# Autodesk Inventor assembly: staw
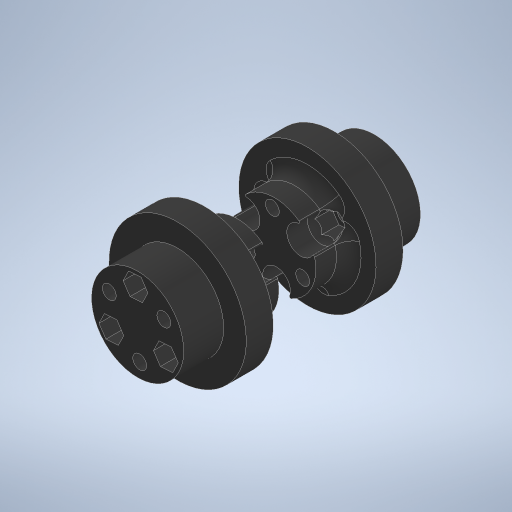
[picture p0: Inventor's stored thumbnail of the model, 512x512]
Saved by Autodesk Inventor 2023 (Build 270158000, 158)
## iProperties
Created: 2023-04-06
Part Number: staw
Document SubType Name: Assembly
Designer: Kamil
Author: Kamil
## Documents named in this file (5)
- C:\Users\Kamil\Desktop\PULPIT\KONARM_2\czlon 3\staw.iam
- C:\Users\Kamil\Desktop\PULPIT\KONARM_2\czlon 3\Os.ipt
- C:\Users\Kamil\Desktop\PULPIT\KONARM_2\czlon 3\Os_lewa.ipt
- C:\Users\Kamil\Desktop\PULPIT\KONARM_2\czlon 3\kółko.ipt
- C:\Users\Kamil\Desktop\PULPIT\KONARM_2\czlon 3\ball bearing(6006).ipt
## Components (6 placed, 4 different names)
1. Os:1 — Zestawiające:1, Zestawiające:2, Zestawiające:3, Zestawiające:12, Zestawiające:13, Zestawiające:15
2. Os_lewa:1 — Zestawiające:1, Zestawiające:2, Zestawiające:3, Zestawiające:10, Zestawiające:11, Zestawiające:16
3. ball bearing(6006):1 — Zestawiające:10, Zestawiające:11, Zestawiające:17
4. ball bearing(6006):2 — Zestawiające:12, Zestawiające:13, Zestawiające:14
5. kółko:2 — Zestawiające:16, Zestawiające:17
6. kółko:3 — Zestawiające:14, Zestawiające:15
## Relationships (11: Mate 11)
- Zestawiające:1 [Mate] (12 mm): Os:1 ↔ Os_lewa:1
- Zestawiające:2 [Mate]: Os:1 ↔ Os_lewa:1
- Zestawiające:3 [Mate]: Os:1 ↔ Os_lewa:1
- Zestawiające:10 [Mate]: Os_lewa:1 ↔ ball bearing(6006):1
- Zestawiające:11 [Mate]: Os_lewa:1 ↔ ball bearing(6006):1
- Zestawiające:12 [Mate]: Os:1 ↔ ball bearing(6006):2
- Zestawiające:13 [Mate]: Os:1 ↔ ball bearing(6006):2
- Zestawiające:14 [Mate]: ball bearing(6006):2 ↔ kółko:3
- Zestawiające:15 [Mate]: Os:1 ↔ kółko:3
- Zestawiające:16 [Mate]: Os_lewa:1 ↔ kółko:2
- Zestawiające:17 [Mate]: ball bearing(6006):1 ↔ kółko:2
